# Autodesk Inventor assembly: Assembly3
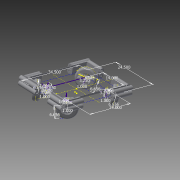
[picture p0: Inventor's stored thumbnail of the model, 180x180]
Saved by Autodesk Inventor 2015 (Build 190159000, 159)
## iProperties
Created: 2016-01-18
Part Number: Assembly3
Document SubType Name: Assembly
Designer: sethbattis
Author: sethbattis
## Documents named in this file (4)
- \\area51\team3566\cad\FRC 2016\Space Claims.iam
- \\area51\team3566\cad\FRC 2016\Basic Frame.ipt
- \\area51\team3566\cad\FRC 2016\Corner Bumper.ipt
- \\area51\team3566\cad\FRC 2016\Wheel Orientation.iam
## Components (6 placed, 3 different names)
1. Basic Frame:1 — Flush:1, Flush:2, Flush:3, Flush:4, Mate:1, Mate:2, Mate:3, Mate:4, Mate:5, Mate:6, Mate:7, Mate:8, Flush:5, Flush:6
2. Wheel Orientation:1 [sub-assembly] — Flush:5, Flush:6
3. Corner Bumper:1 — Flush:3, Mate:1, Mate:2
4. Corner Bumper:2 — Flush:1, Mate:5, Mate:6
5. Corner Bumper:3 — Flush:2, Mate:7, Mate:8
6. Corner Bumper:4 — Flush:4, Mate:3, Mate:4
## Relationships (14: Mate 8, Flush 6)
- Flush:1: Basic Frame:1 ↔ Corner Bumper:2
- Flush:2: Basic Frame:1 ↔ Corner Bumper:3
- Flush:3: Basic Frame:1 ↔ Corner Bumper:1
- Flush:4: Basic Frame:1 ↔ Corner Bumper:4
- Mate:1: Basic Frame:1 ↔ Corner Bumper:1
- Mate:2: Basic Frame:1 ↔ Corner Bumper:1
- Mate:3: Basic Frame:1 ↔ Corner Bumper:4
- Mate:4: Basic Frame:1 ↔ Corner Bumper:4
- Mate:5: Basic Frame:1 ↔ Corner Bumper:2
- Mate:6: Basic Frame:1 ↔ Corner Bumper:2
- Mate:7: Basic Frame:1 ↔ Corner Bumper:3
- Mate:8: Basic Frame:1 ↔ Corner Bumper:3
- Flush:5: Basic Frame:1 ↔ Wheel Orientation:1
- Flush:6: Basic Frame:1 ↔ Wheel Orientation:1
